# Autodesk Inventor assembly: B3M-SC-1170-A_with_ClampHorn
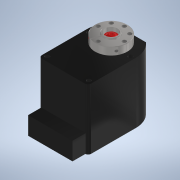
[picture p0: Inventor's stored thumbnail of the model, 180x180]
Saved by Autodesk Inventor 2020.4 (Build 244396000, 396)
## iProperties
Created: 2022-03-18
Part Number: B3M-SC-1170-A_with_ClampHorn
Document SubType Name: Assembly
Designer: MasatoKubotera
Author: MasatoKubotera
## Documents named in this file (3)
- C:\Users\Masato\Documents\Inventor\CIT Brains_Inventor\SUSTAINA-OP\ReadyMade\KONDO\B3M-SC-1170-A_with_ClampHorn.iam
- C:\Users\Masato\Documents\Inventor\CIT Brains_Inventor\SUSTAINA-OP\ReadyMade\KONDO\B3M-SC-1170-A.ipt
- C:\Users\Masato\Documents\Inventor\CIT Brains_Inventor\SUSTAINA-OP\ReadyMade\KONDO\ClampHorn.iam
## Components (2 placed, 2 different names)
1. B3M-SC-1170-A:1 — 挿入:1, メイト:1, メイト:2, メイト:3, 角度:1
2. ClampHorn:1 [sub-assembly] — 挿入:1, 角度:1
## Relationships (5: Mate 3, Insert 1, Angle 1)
- 挿入:1 [Insert]: B3M-SC-1170-A:1 ↔ ClampHorn:1
- メイト:1 [Mate]: B3M-SC-1170-A:1
- メイト:2 [Mate]: B3M-SC-1170-A:1
- メイト:3 [Mate]: B3M-SC-1170-A:1
- 角度:1 [Angle] (0 deg): B3M-SC-1170-A:1 ↔ ClampHorn:1
